# Autodesk Inventor assembly: ZcolumAssy
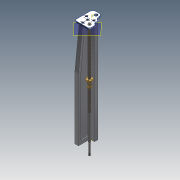
[picture p0: Inventor's stored thumbnail of the model, 180x180]
Saved by Autodesk Inventor 2019 (Build 230136000, 136)
## iProperties
Created: 2019-01-01
Part Number: ZcolumAssy
Document SubType Name: Assembly
Designer: LillaHunden
Mass: 1739.88 g
Surface Area: 1825.2 cm^2
Volume: 553.34 cm^3
Density: 3.14432 g/cm^3
Author: LillaHunden
## Documents named in this file (12)
- C:\Users\LillaHunden\Documents\Inventor\3dprinter\3dPrinter\ZcolumAssy.iam
- C:\Users\LillaHunden\Documents\Inventor\3dprinter\3dPrinter\Zcolumn.ipt
- C:\Users\LillaHunden\Documents\Inventor\3dprinter\3dPrinter\ZcolStiffer.ipt
- C:\Users\LillaHunden\Documents\Inventor\3dprinter\3dPrinter\Linear Rials import\Rail Z.ipt
- C:\Users\LillaHunden\Documents\Inventor\3dprinter\3dPrinter\ZBaringBracket.ipt
- C:\Users\LillaHunden\Documents\Inventor\3dprinter\3dPrinter\Linear Rials import\MGN block.iam
- C:\Users\LillaHunden\Documents\Inventor\3dprinter\3dPrinter\Trapezoidal lead screw tr8x8-4 Z.ipt
- C:\Users\LillaHunden\Documents\Inventor\3dprinter\3dPrinter\Linear Rials import\TR8_8(P4) Antibacklash Nut w. spring.ipt
- C:\Users\LillaHunden\Documents\Inventor\3dprinter\3dPrinter\FR168ZZ flangde bearing.ipt
- C:\Users\LillaHunden\Documents\Inventor\3dprinter\3dPrinter\ZcolumAssy\Design Accelerator\Bolted Connection1.iam
- C:\Users\LillaHunden\Documents\Inventor\3dprinter\3dPrinter\ZcolumAssy\Design Accelerator\Bolted Connection2.iam
- C:\Users\LillaHunden\Documents\Inventor\3dprinter\3dPrinter\ZcolumAssy\Design Accelerator\Bolted Connection3.iam
## Components (13 placed, 9 different names)
1. Zcolumn:2 — Mate:1, Flush:1, Mate:2, Flush:2, Mate:12, Mate:13, Flush:3, Mate:21
2. ZcolStiffer:1 — Mate:1, Flush:1, Mate:2, Mate:5, Mate:6, Mate:7
3. Rail Z:1 — Mate:12, Mate:13, Flush:3, Mate:14, Mate:15, Mate:16, Mate:17
4. ZBaringBracket:1 — Mate:5, Mate:6, Mate:7, Flush:2, Mate:8, Mate:9, Mate:20, Mate:22, Mate:23, Mate:25, Mate:26
5. MGN block:1 [sub-assembly] — Mate:16, Mate:17, Flush:4, Flush:5
6. MGN block:2 [sub-assembly] — Flush:4, Flush:5
7. Trapezoidal lead screw tr8x8-4 Z:1 — Mate:10, Mate:11, Mate:24
8. TR8_8(P4) Antibacklash Nut w. spring:1 — Mate:24
9. FR168ZZ flangde bearing:1 — Mate:8, Mate:9, Mate:10, Mate:11
10. Bolted Connection:1 [sub-assembly] — Mate:14, Mate:15
11. Bolted Connection:2 [sub-assembly] — Mate:22, Mate:23
12. Bolted Connection:3 [sub-assembly] — Mate:20, Mate:21
13. FR168ZZ flangde bearing:2 — Mate:25, Mate:26
## Relationships (27: Mate 22, Flush 5)
- Mate:1: Zcolumn:2 ↔ ZcolStiffer:1
- Flush:1: Zcolumn:2 ↔ ZcolStiffer:1
- Mate:2: Zcolumn:2 ↔ ZcolStiffer:1
- Mate:5: ZcolStiffer:1 ↔ ZBaringBracket:1
- Mate:6: ZcolStiffer:1 ↔ ZBaringBracket:1
- Mate:7: ZcolStiffer:1 ↔ ZBaringBracket:1
- Flush:2: Zcolumn:2 ↔ ZBaringBracket:1
- Mate:8: ZBaringBracket:1 ↔ FR168ZZ flangde bearing:1
- Mate:9: ZBaringBracket:1 ↔ FR168ZZ flangde bearing:1
- Mate:10: Trapezoidal lead screw tr8x8-4 Z:1 ↔ FR168ZZ flangde bearing:1
- Mate:11: Trapezoidal lead screw tr8x8-4 Z:1 ↔ FR168ZZ flangde bearing:1
- Mate:12: Zcolumn:2 ↔ Rail Z:1
- Mate:13: Zcolumn:2 ↔ Rail Z:1
- Flush:3 (5 mm): Zcolumn:2 ↔ Rail Z:1
- Mate:14: Rail Z:1 ↔ Bolted Connection:1
- Mate:15: Rail Z:1 ↔ Bolted Connection:1
- Mate:16: Rail Z:1 ↔ MGN block:1
- Mate:17: Rail Z:1 ↔ MGN block:1
- Flush:4: MGN block:1 ↔ MGN block:2
- Flush:5: MGN block:1 ↔ MGN block:2
- Mate:20: ZBaringBracket:1 ↔ Bolted Connection:3
- Mate:21: Zcolumn:2 ↔ Bolted Connection:3
- Mate:22: ZBaringBracket:1 ↔ Bolted Connection:2
- Mate:23: ZBaringBracket:1 ↔ Bolted Connection:2
- Mate:24: Trapezoidal lead screw tr8x8-4 Z:1 ↔ TR8_8(P4) Antibacklash Nut w. spring:1
- Mate:25: ZBaringBracket:1 ↔ FR168ZZ flangde bearing:2
- Mate:26: ZBaringBracket:1 ↔ FR168ZZ flangde bearing:2
